# Autodesk Inventor assembly: Clamping Block
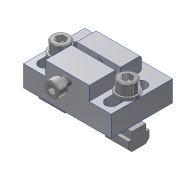
[picture p0: Inventor's stored thumbnail of the model, 180x180]
Saved by Autodesk Inventor 2016 (Build 200138000, 138)
## iProperties
Created: 2015-08-18
Part Number: Clamping Block
Document SubType Name: Assembly
## Documents named in this file (7)
- E:\GitHub\CNC-Router_Accessories\Clamping Block Assembly.iam
- E:\GitHub\Buy-Parts\T-Nutenstein 8 - M6_St.ipt
- E:\GitHub\Standard-Parts\U-Scheibe_ISO 7089 - 6 - 140 HV_St-Vzkt.ipt
- E:\GitHub\CNC-Router_Accessories\Clamping Block.ipt
- E:\GitHub\CNC-Router_Accessories\Jaw.ipt
- E:\GitHub\Standard-Parts\Zyl-Schr_ISO 4762 - M5 x 25_St-Vzkt.ipt
- E:\GitHub\Standard-Parts\Zyl-Schr_ISO 4762 - M6 x 20_St-Vzkt.ipt
## Components (9 placed, 6 different names)
1. Clamping Block:1 — Mate:1, Mate:2, Mate:3, Mate:4, Mate:5, Mate:8, Mate:9, Mate:10, Mate:12, Angle:1
2. T-Nutenstein 8 - M6_St:1 — Flush:1, Flush:2, Mate:1, Mate:3, Mate:7, Angle:1
3. T-Nutenstein 8 - M6_St:2 — Flush:1, Flush:2, Mate:2, Mate:6
4. Zyl-Schr_ISO 4762 - M6 x 20_St-Vzkt:1 — Insert:1, Mate:6
5. U-Scheibe_ISO 7089 - 6 - 140 HV_St-Vzkt:1 — Insert:1, Mate:5
6. Zyl-Schr_ISO 4762 - M6 x 20_St-Vzkt:2 — Mate:7, Mate:12
7. U-Scheibe_ISO 7089 - 6 - 140 HV_St-Vzkt:2 — Mate:4
8. Jaw:1 — Mate:8, Mate:9, Mate:11
9. Zyl-Schr_ISO 4762 - M5 x 25_St-Vzkt:1 — Mate:10, Mate:11
## Relationships (17: Mate 12, Flush 2, Insert 2, Angle 1)
- Flush:1: T-Nutenstein 8 - M6_St:1 ↔ T-Nutenstein 8 - M6_St:2
- Flush:2: T-Nutenstein 8 - M6_St:1 ↔ T-Nutenstein 8 - M6_St:2
- Mate:1 (-6 mm): Clamping Block:1 ↔ T-Nutenstein 8 - M6_St:1
- Mate:2 (-6 mm): Clamping Block:1 ↔ T-Nutenstein 8 - M6_St:2
- Mate:3 (6 mm): Clamping Block:1 ↔ T-Nutenstein 8 - M6_St:1
- Insert:1: Zyl-Schr_ISO 4762 - M6 x 20_St-Vzkt:1 ↔ U-Scheibe_ISO 7089 - 6 - 140 HV_St-Vzkt:1
- [Insert]: Zyl-Schr_ISO 4762 - M6 x 20_St-Vzkt:2 ↔ U-Scheibe_ISO 7089 - 6 - 140 HV_St-Vzkt:2
- Mate:4: Clamping Block:1 ↔ U-Scheibe_ISO 7089 - 6 - 140 HV_St-Vzkt:2
- Mate:5: Clamping Block:1 ↔ U-Scheibe_ISO 7089 - 6 - 140 HV_St-Vzkt:1
- Mate:6: T-Nutenstein 8 - M6_St:2 ↔ Zyl-Schr_ISO 4762 - M6 x 20_St-Vzkt:1
- Mate:7: T-Nutenstein 8 - M6_St:1 ↔ Zyl-Schr_ISO 4762 - M6 x 20_St-Vzkt:2
- Mate:8: Clamping Block:1 ↔ Jaw:1
- Mate:9: Clamping Block:1 ↔ Jaw:1
- Mate:10: Clamping Block:1 ↔ Zyl-Schr_ISO 4762 - M5 x 25_St-Vzkt:1
- Mate:11: Jaw:1 ↔ Zyl-Schr_ISO 4762 - M5 x 25_St-Vzkt:1
- Mate:12 (-6 mm): Clamping Block:1 ↔ Zyl-Schr_ISO 4762 - M6 x 20_St-Vzkt:2
- Angle:1 (0 deg): Clamping Block:1 ↔ T-Nutenstein 8 - M6_St:1
## Named parameters: d13_d12 = 0 mm
